# Autodesk Inventor assembly: Epsilon grabbers 2
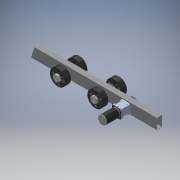
[picture p0: Inventor's stored thumbnail of the model, 180x180]
Saved by Autodesk Inventor 2019 (Build 230136000, 136)
## iProperties
Created: 2019-03-06
Part Number: Epsilon grabbers 2
Document SubType Name: Assembly
Designer: josh
Author: josh
## Documents named in this file (6)
- D:\Synthesis Robots\Epsilon\Epsilon Grabbers\Epsilon grabbers 2.iam
- D:\Synthesis Robots\Epsilon\Epsilon Grabbers\Aluminum Channel Arm.ipt
- D:\Synthesis Robots\Epsilon\Epsilon Grabbers\Bag Motor parts\VersaPlanetary_v1_Single_Stage_10_1_with_BAG.iam
- D:\Synthesis Robots\Epsilon\Epsilon Grabbers\am-0646 S25-22HA-500 Hex Sprocket.ipt
- D:\Synthesis Robots\Epsilon\Epsilon Grabbers\Grabbing unit\Eplison gripper 1.iam
- D:\Synthesis Robots\Epsilon\Epsilon Grabbers\Grabbing unit\Epsilon gripper 2.iam
## Components (5 placed, 5 different names)
1. Aluminum Channel Arm:1 — Mate:1, Mate:2, Mate:5, Tangent:1, Tangent:2, Mate:6, Tangent:3, Tangent:4, Mate:7
2. VersaPlanetary_v1_Single_Stage_10_1_with_BAG:1 [sub-assembly] — Mate:1, Mate:2, Mate:3, Mate:4
3. am-0646 S25-22HA-500 Hex Sprocket:1 — Mate:3, Mate:4, Mate:5
4. Eplison gripper 1:1 [sub-assembly] — Tangent:1, Tangent:2, Mate:6
5. Epsilon gripper 2:1 [sub-assembly] — Tangent:3, Tangent:4, Mate:7
## Relationships (11: Mate 7, Tangent 4)
- Mate:1: Aluminum Channel Arm:1 ↔ VersaPlanetary_v1_Single_Stage_10_1_with_BAG:1
- Mate:2: Aluminum Channel Arm:1 ↔ VersaPlanetary_v1_Single_Stage_10_1_with_BAG:1
- Mate:3: VersaPlanetary_v1_Single_Stage_10_1_with_BAG:1 ↔ am-0646 S25-22HA-500 Hex Sprocket:1
- Mate:4: VersaPlanetary_v1_Single_Stage_10_1_with_BAG:1 ↔ am-0646 S25-22HA-500 Hex Sprocket:1
- Mate:5: Aluminum Channel Arm:1 ↔ am-0646 S25-22HA-500 Hex Sprocket:1
- Tangent:1: Aluminum Channel Arm:1 ↔ Eplison gripper 1:1
- Tangent:2: Aluminum Channel Arm:1 ↔ Eplison gripper 1:1
- Mate:6: Aluminum Channel Arm:1 ↔ Eplison gripper 1:1
- Tangent:3: Aluminum Channel Arm:1 ↔ Epsilon gripper 2:1
- Tangent:4: Aluminum Channel Arm:1 ↔ Epsilon gripper 2:1
- Mate:7: Aluminum Channel Arm:1 ↔ Epsilon gripper 2:1
